# Autodesk Inventor assembly: shaft coupling assembly
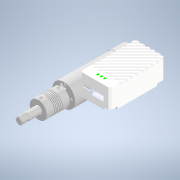
[picture p0: Inventor's stored thumbnail of the model, 180x180]
Saved by Autodesk Inventor 2021.1 (Build 251245000, 245)
## iProperties
Created: 2020-08-21
Part Number: shaft coupling assembly
Document SubType Name: Assembly
Designer: Alex
Author: Alex
## Documents named in this file (5)
- C:\Users\Public\Documents\Autodesk\Inventor 2021\shaft coupling assembly.iam
- C:\Users\Public\Documents\Autodesk\Inventor 2021\flexible shaft coupling.ipt
- C:\Users\Public\Documents\Autodesk\Inventor 2021\cut quarter inch extension.ipt
- C:\Users\Public\Documents\Autodesk\Inventor 2021\Allen_Motor_3D.ipt
- C:\Users\Public\Documents\Autodesk\Inventor 2021\micro controller.ipt
## Components (4 placed, 4 different names)
1. flexible shaft coupling:1 — Cylindrical:1, Rotational:1
2. cut quarter inch extension:1 — Cylindrical:1
3. Allen_Motor_3D:1 — Rotational:1
4. micro controller:1
## Relationships (2: CylindricalJoint 1, RevoluteJoint 1)
- Cylindrical:1: flexible shaft coupling:1 ↔ cut quarter inch extension:1
- Rotational:1 [RevoluteJoint]: flexible shaft coupling:1 ↔ Allen_Motor_3D:1
